# Autodesk Inventor assembly: Rahmen
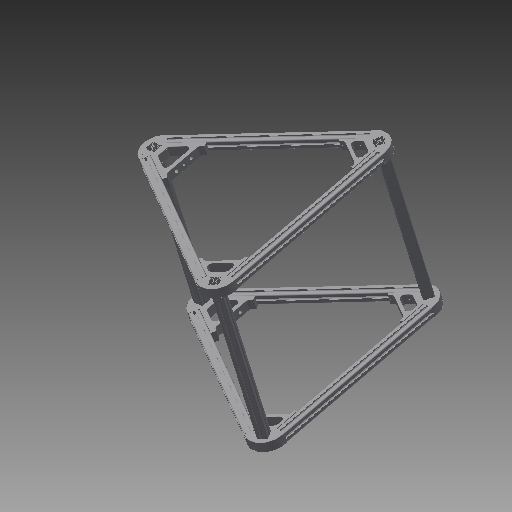
[picture p0: Inventor's stored thumbnail of the model, 512x512]
Saved by Autodesk Inventor 2019 (Build 230136000, 136)
## iProperties
Created: 2018-08-17
Part Number: Rahmen
Document SubType Name: Assembly
Designer: Julia
Author: Julia
## Documents named in this file (4)
- C:\Users\Julia\Documents\Inventor\3D_Drucker_v01\Rahmen.iam
- C:\Users\Julia\Documents\Inventor\3D_Drucker_v01\Profil_Winkel.ipt
- C:\Users\Julia\Documents\Inventor\3D_Drucker_v01\Alu_Proil_40.ipt
- C:\Users\Julia\Documents\Inventor\3D_Drucker_v01\Profil_Winkel_oben.ipt
## Components (15 placed, 3 different names)
1. Alu_Proil_40:1 — Mate:7, Mate:8, Mate:31, Mate:32
2. Alu_Proil_40:2 — Mate:5, Mate:6, Mate:33
3. Profil_Winkel:2 — Mate:5, Mate:6, Mate:10, Mate:11, Mate:29, Mate:30, Flush:4
4. Profil_Winkel:3 — Mate:7, Mate:8, Mate:9, Mate:25, Mate:26, Mate:31
5. Alu_Proil_40:3 — Mate:9, Mate:10, Mate:11
6. Alu_Proil_40:4 — Mate:35, Mate:36
7. Alu_Proil_40:5 — Mate:34
8. Profil_Winkel:5
9. Profil_Winkel:6 — Mate:23, Mate:24, Flush:3, Mate:35
10. Alu_Proil_40:6
11. Alu_Proil_40:7 — Mate:23, Mate:24, Mate:25, Mate:26, Flush:3
12. Alu_Proil_40:8 — Mate:37
13. Alu_Proil_40:9 — Mate:29, Mate:30, Flush:4
14. Profil_Winkel_oben:1 — Mate:32, Mate:33
15. Profil_Winkel_oben:2 — Mate:34, Mate:36, Mate:37
## Relationships (29: Mate 27, Flush 2)
- Mate:5: Alu_Proil_40:2 ↔ Profil_Winkel:2
- Mate:6: Alu_Proil_40:2 ↔ Profil_Winkel:2
- Mate:7: Alu_Proil_40:1 ↔ Profil_Winkel:3
- Mate:8: Alu_Proil_40:1 ↔ Profil_Winkel:3
- Mate:9: Profil_Winkel:3 ↔ Alu_Proil_40:3
- Mate:10: Profil_Winkel:2 ↔ Alu_Proil_40:3
- Mate:11: Profil_Winkel:2 ↔ Alu_Proil_40:3
- [Mate]: Alu_Proil_40:5 ↔ Profil_Winkel:5
- [Mate]: Alu_Proil_40:5 ↔ Profil_Winkel:5
- [Mate]: Alu_Proil_40:4 ↔ Profil_Winkel:6
- [Mate]: Alu_Proil_40:4 ↔ Profil_Winkel:6
- [Mate]: Profil_Winkel:6 ↔ Alu_Proil_40:6
- [Mate]: Profil_Winkel:5 ↔ Alu_Proil_40:6
- [Mate]: Profil_Winkel:5 ↔ Alu_Proil_40:6
- Mate:23: Profil_Winkel:6 ↔ Alu_Proil_40:7
- Mate:24: Profil_Winkel:6 ↔ Alu_Proil_40:7
- Mate:25: Profil_Winkel:3 ↔ Alu_Proil_40:7
- Mate:26: Profil_Winkel:3 ↔ Alu_Proil_40:7
- Flush:3: Profil_Winkel:6 ↔ Alu_Proil_40:7
- Mate:29: Profil_Winkel:2 ↔ Alu_Proil_40:9
- Mate:30: Profil_Winkel:2 ↔ Alu_Proil_40:9
- Flush:4: Profil_Winkel:2 ↔ Alu_Proil_40:9
- Mate:31: Alu_Proil_40:1 ↔ Profil_Winkel:3
- Mate:32: Alu_Proil_40:1 ↔ Profil_Winkel_oben:1
- Mate:33: Alu_Proil_40:2 ↔ Profil_Winkel_oben:1
- Mate:34: Alu_Proil_40:5 ↔ Profil_Winkel_oben:2
- Mate:35: Alu_Proil_40:4 ↔ Profil_Winkel:6
- Mate:36: Alu_Proil_40:4 ↔ Profil_Winkel_oben:2
- Mate:37: Alu_Proil_40:8 ↔ Profil_Winkel_oben:2
## Named parameters: d12_d4 = 0 mm, d13_d5 = 0 mm, d14_d6 = 0 mm, d15_d7 = 0 mm, d16_d8 = 0 mm, d17_d9 = 0 mm, d18_d10 = 0 mm
